# Autodesk Inventor assembly: NucPower
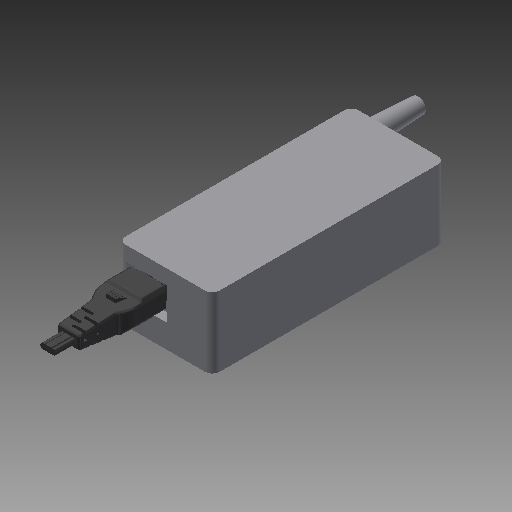
[picture p0: Inventor's stored thumbnail of the model, 512x512]
Saved by Autodesk Inventor 2019 (Build 230136000, 136)
## iProperties
Created: 2019-05-22
Part Number: NucPower
Document SubType Name: Assembly
Designer: Jorian Bruslind
Author: Jorian Bruslind
## Documents named in this file (3)
- E:\Downloads\Robot_Controller_Models\NUC5CPYH-NUC5PPYH-CHASSIS-STEP\NucPower.iam
- E:\Downloads\Robot_Controller_Models\NUC5CPYH-NUC5PPYH-CHASSIS-STEP\NucPowerBrick.ipt
- E:\Downloads\Robot_Controller_Models\connector-3-prong-iec-320-c-5-1.snapshot.2\IEC 320 C-5.ipt
## Components (2 placed, 2 different names)
1. NucPowerBrick:1 — Mate:1, Mate:2, Mate:3
2. IEC 320 C-5:1 — Mate:1, Mate:2, Mate:3
## Relationships (3: Mate 3)
- Mate:1: NucPowerBrick:1 ↔ IEC 320 C-5:1
- Mate:2 (1 mm): NucPowerBrick:1 ↔ IEC 320 C-5:1
- Mate:3 (1 mm): NucPowerBrick:1 ↔ IEC 320 C-5:1
